# Autodesk Inventor assembly: Robot
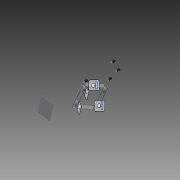
[picture p0: Inventor's stored thumbnail of the model, 180x180]
Saved by Autodesk Inventor 2014 (Build 180170000, 170)
## iProperties
Created: 2014-01-21
Part Number: Robot
Document SubType Name: Assembly
Designer: NilesStanton
Author: NilesStanton
## Documents named in this file (7)
- C:\GitHub\team3566-2014\CAD\Robot.iam
- C:\FIRST-2014-KOP\Drive Base Kit\2014 Sidings.ipt
- C:\FIRST-2014-KOP\Motors\MOT_CIM-Motor_217-2000.iam
- C:\FIRST-2014-KOP\Additions\Flat Board.ipt
- C:\FIRST-2014-KOP\Additions\Front Paneling.ipt
- C:\FIRST-2014-KOP\Additions\3.5 in spacer.ipt
- C:\FIRST-2014-KOP\Additions\Mechanum Wheel.ipt
## Components (18 placed, 6 different names)
1. 2014 Sidings:1 — Flush:8, Mate:4, Angle:5
2. 2014 Sidings:2 — Mate:3, Flush:3, Angle:3, Flush:11, Flush:14, Flush:15
3. MOT_CIM-Motor_217-2000:1 [sub-assembly]
4. MOT_CIM-Motor_217-2000:2 [sub-assembly]
5. MOT_CIM-Motor_217-2000:3 [sub-assembly]
6. MOT_CIM-Motor_217-2000:4 [sub-assembly]
7. Flat Board:1
8. 2014 Sidings:3
9. Front Paneling:1 — Mate:2, Flush:2, Angle:2, Mate:3, Flush:3, Angle:3
10. Front Paneling:2 — Mate:1, Flush:1, Angle:1, Flush:5, Flush:7, Flush:9, Flush:10
11. 3.5 in spacer:1 — Flush:9, Flush:10, Flush:11, Flush:12, Flush:13, Mate:5, Angle:6, Tangent:1, Tangent:2
12. 3.5 in spacer:2 — Flush:5, Flush:6, Angle:4, Flush:7, Flush:8, Mate:4, Angle:5, Tangent:3, Tangent:4
13. 2014 Sidings:4 — Flush:12, Flush:13, Mate:5, Angle:6
14. 2014 Sidings:5 — Mate:1, Flush:1, Angle:1, Mate:2, Flush:2, Angle:2, Flush:6, Angle:4, Flush:16, Flush:17
15. Mechanum Wheel:1 — Flush:14, Tangent:1
16. Mechanum Wheel:2 — Flush:17, Tangent:4
17. Mechanum Wheel:3 — Flush:15, Tangent:2
18. Mechanum Wheel:4 — Flush:16, Tangent:3
## Relationships (31: Flush 16, Angle 6, Mate 5, Tangent 4)
- Mate:1: Front Paneling:2 ↔ 2014 Sidings:5
- Flush:1: Front Paneling:2 ↔ 2014 Sidings:5
- Angle:1 (90 deg): Front Paneling:2 ↔ 2014 Sidings:5
- Mate:2: Front Paneling:1 ↔ 2014 Sidings:5
- Flush:2: Front Paneling:1 ↔ 2014 Sidings:5
- Angle:2 (90 deg): Front Paneling:1 ↔ 2014 Sidings:5
- Mate:3: 2014 Sidings:2 ↔ Front Paneling:1
- Flush:3: 2014 Sidings:2 ↔ Front Paneling:1
- Angle:3 (90 deg): 2014 Sidings:2 ↔ Front Paneling:1
- Flush:5: Front Paneling:2 ↔ 3.5 in spacer:2
- Flush:6: 3.5 in spacer:2 ↔ 2014 Sidings:5
- Angle:4 (90 deg): 3.5 in spacer:2 ↔ 2014 Sidings:5
- Flush:7: Front Paneling:2 ↔ 3.5 in spacer:2
- Flush:8: 2014 Sidings:1 ↔ 3.5 in spacer:2
- Mate:4: 2014 Sidings:1 ↔ 3.5 in spacer:2
- Angle:5 (90 deg): 2014 Sidings:1 ↔ 3.5 in spacer:2
- Flush:9: Front Paneling:2 ↔ 3.5 in spacer:1
- Flush:10: Front Paneling:2 ↔ 3.5 in spacer:1
- Flush:11: 2014 Sidings:2 ↔ 3.5 in spacer:1
- Flush:12: 3.5 in spacer:1 ↔ 2014 Sidings:4
- Flush:13: 3.5 in spacer:1 ↔ 2014 Sidings:4
- Mate:5: 3.5 in spacer:1 ↔ 2014 Sidings:4
- Angle:6 (90 deg): 3.5 in spacer:1 ↔ 2014 Sidings:4
- Flush:14: 2014 Sidings:2 ↔ Mechanum Wheel:1
- Flush:15: 2014 Sidings:2 ↔ Mechanum Wheel:3
- Tangent:1 (50.8 mm): 3.5 in spacer:1 ↔ Mechanum Wheel:1
- Tangent:2 (622.3 mm): 3.5 in spacer:1 ↔ Mechanum Wheel:3
- Flush:16: 2014 Sidings:5 ↔ Mechanum Wheel:4
- Flush:17: 2014 Sidings:5 ↔ Mechanum Wheel:2
- Tangent:3 (50.8 mm): 3.5 in spacer:2 ↔ Mechanum Wheel:4
- Tangent:4 (622.3 mm): 3.5 in spacer:2 ↔ Mechanum Wheel:2
